# Autodesk Inventor assembly: Arm Assembly
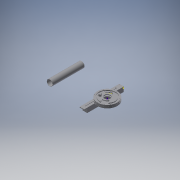
[picture p0: Inventor's stored thumbnail of the model, 180x180]
Saved by Autodesk Inventor 2016 (Build 200138000, 138)
## iProperties
Created: 2016-04-23
Part Number: Arm Assembly
Document SubType Name: Assembly
Designer: rubenjm
Author: rubenjm
## Documents named in this file (22)
- C:\Users\rubenjm\Documents\To Transfer\2k16 Spring\RME\GGC\V3\Arm Assembly.iam
- C:\Users\rubenjm\Documents\To Transfer\2k16 Spring\RME\GGC\V3\Inner Pole.ipt
- C:\Users\rubenjm\Documents\To Transfer\2k16 Spring\RME\GGC\V3\Arm Base.ipt
- C:\Users\rubenjm\Documents\To Transfer\2k16 Spring\RME\GGC\V3\Holder.ipt
- C:\Users\rubenjm\Documents\To Transfer\2k16 Spring\RME\GGC\V3\Threaded Rod Nut.ipt
- C:\Users\rubenjm\Documents\To Transfer\2k16 Spring\RME\GGC\V3\Unthreaded Rod.ipt
- C:\Users\rubenjm\Documents\To Transfer\2k16 Spring\RME\GGC\V3\Threaded Rod.ipt
- C:\Users\rubenjm\Documents\To Transfer\2k16 Spring\RME\GGC\V3\NEMA23 Motor.ipt
- C:\Users\rubenjm\Documents\To Transfer\2k16 Spring\RME\GGC\V3\Motor Coupler.ipt
- C:\Users\rubenjm\Documents\To Transfer\2k16 Spring\RME\GGC\V3\Far End Cap.ipt
- C:\Users\rubenjm\Documents\To Transfer\2k16 Spring\RME\GGC\V3\Near Holder.ipt
- C:\Users\rubenjm\Documents\To Transfer\2k16 Spring\RME\GGC\V3\Motor Bracket.ipt
- C:\Users\rubenjm\Documents\To Transfer\2k16 Spring\RME\GGC\V3\Near End Cap.ipt
- C:\Users\rubenjm\Documents\To Transfer\2k16 Spring\RME\GGC\V3\Arm Side.ipt
- C:\Users\rubenjm\Documents\To Transfer\2k16 Spring\RME\GGC\V3\Arm Top.ipt
- C:\Users\rubenjm\Documents\To Transfer\2k16 Spring\RME\GGC\V3\Turntable Top.ipt
- C:\Users\rubenjm\Documents\To Transfer\2k16 Spring\RME\GGC\V3\Turntable.ipt
- C:\Users\rubenjm\Documents\To Transfer\2k16 Spring\RME\GGC\V3\Turntable Ring Gear.iam
- C:\Users\rubenjm\Documents\To Transfer\2k16 Spring\RME\GGC\V3\Turntable Sheath.ipt
- C:\Users\rubenjm\Documents\To Transfer\2k16 Spring\RME\GGC\V3\NEMA16 Motor.ipt
- C:\Users\rubenjm\Documents\To Transfer\2k16 Spring\RME\GGC\V3\Turntable Mount.ipt
- C:\Users\rubenjm\Documents\To Transfer\2k16 Spring\RME\GGC\V3\Inner Gear.iam
## Components (28 placed, 21 different names)
1. Inner Pole:1
2. Arm Base:1 — Mate:1, Mate:2, Mate:15, Mate:26, Mate:27, Flush:1, Flush:3, Mate:34, Mate:38, Flush:4, Mate:40, Flush:5, Mate:41, Mate:42, Mate:43, Flush:6, Flush:7, Flush:9, Flush:11, Mate:48
3. Holder:1 — Mate:1, Mate:2, Mate:8, Mate:9, Mate:10, Mate:12, Mate:13, Mate:49
4. Holder:2 — Mate:15, Mate:16, Mate:17, Mate:18, Mate:19, Mate:20, Mate:46, Mate:47, Mate:51
5. Threaded Rod Nut:1 — Mate:8, Mate:9, Mate:10, Mate:11
6. Threaded Rod Nut:2 — Mate:18, Mate:19, Mate:20
7. Unthreaded Rod:1 — Mate:13, Mate:16, Mate:28
8. Unthreaded Rod:2 — Mate:12, Mate:17, Mate:29
9. Threaded Rod:1 — Mate:11, Mate:24, Mate:25, Mate:30
10. NEMA23 Motor:1 — Mate:35, Mate:36, Mate:37, Mate:39
11. Motor Coupler:1 — Mate:24, Mate:25
12. Far End Cap:1 — Mate:26, Mate:27, Flush:1, Mate:28, Mate:29, Mate:30, Mate:44, Flush:12
13. Near Holder:1 — Flush:5, Mate:41, Mate:42
14. Motor Bracket:1 — Flush:3, Mate:34, Mate:35, Mate:36, Mate:37, Mate:38
15. Near End Cap:1 — Mate:39, Flush:4, Mate:40, Flush:8, Flush:10
16. Arm Side:1 — Mate:43, Flush:6, Flush:7, Flush:8
17. Arm Side:2 — Flush:9, Flush:10, Flush:11, Mate:45
18. Arm Top:1 — Mate:44, Mate:45, Flush:12
19. Turntable Top:1 — Mate:46, Mate:47, Mate:48, Mate:49, Mate:50, Mate:53
20. Turntable:1 — Mate:60, Mate:61, Mate:62, Mate:69, Mate:70, Mate:71
21. Turntable Top:2 — Mate:50, Mate:51, Mate:53, Mate:54, Mate:55, Mate:56
22. Turntable Ring Gear:1 [sub-assembly] — Mate:54, Mate:55, Mate:56, Mate:57, Mate:58, Mate:59, Mate:62
23. Turntable Ring Gear:2 [sub-assembly] — Mate:57, Mate:58, Mate:59, Mate:60, Mate:61, Mate:63, Mate:64, Mate:65
24. Turntable Sheath:1 — Mate:66, Mate:67, Mate:68
25. Turntable Sheath:2 — Mate:63, Mate:64, Mate:65, Mate:66, Mate:67, Mate:68
26. NEMA16 Motor:1 — Mate:72, Mate:73, Mate:74, Mate:75, Mate:76
27. Turntable Mount:1 — Mate:69, Mate:70, Mate:71, Mate:72, Mate:73, Mate:74
28. Inner Gear:1 [sub-assembly] — Mate:75, Mate:76
## Relationships (74: Mate 63, Flush 11)
- Mate:1: Arm Base:1 ↔ Holder:1
- Mate:2: Arm Base:1 ↔ Holder:1
- Mate:8: Holder:1 ↔ Threaded Rod Nut:1
- Mate:9: Holder:1 ↔ Threaded Rod Nut:1
- Mate:10: Holder:1 ↔ Threaded Rod Nut:1
- Mate:11: Threaded Rod Nut:1 ↔ Threaded Rod:1
- Mate:12: Holder:1 ↔ Unthreaded Rod:2
- Mate:13: Holder:1 ↔ Unthreaded Rod:1
- Mate:15: Arm Base:1 ↔ Holder:2
- Mate:16: Holder:2 ↔ Unthreaded Rod:1
- Mate:17: Holder:2 ↔ Unthreaded Rod:2
- Mate:18: Holder:2 ↔ Threaded Rod Nut:2
- Mate:19: Holder:2 ↔ Threaded Rod Nut:2
- Mate:20: Holder:2 ↔ Threaded Rod Nut:2
- Mate:24: Threaded Rod:1 ↔ Motor Coupler:1
- Mate:25: Threaded Rod:1 ↔ Motor Coupler:1
- Mate:26: Arm Base:1 ↔ Far End Cap:1
- Mate:27: Arm Base:1 ↔ Far End Cap:1
- Flush:1: Arm Base:1 ↔ Far End Cap:1
- Mate:28: Unthreaded Rod:1 ↔ Far End Cap:1
- Mate:29: Unthreaded Rod:2 ↔ Far End Cap:1
- Mate:30: Threaded Rod:1 ↔ Far End Cap:1
- Flush:3: Arm Base:1 ↔ Motor Bracket:1
- Mate:34: Arm Base:1 ↔ Motor Bracket:1
- Mate:35: NEMA23 Motor:1 ↔ Motor Bracket:1
- Mate:36: NEMA23 Motor:1 ↔ Motor Bracket:1
- Mate:37: NEMA23 Motor:1 ↔ Motor Bracket:1
- Mate:38: Arm Base:1 ↔ Motor Bracket:1
- Mate:39: NEMA23 Motor:1 ↔ Near End Cap:1
- Flush:4: Arm Base:1 ↔ Near End Cap:1
- Mate:40: Arm Base:1 ↔ Near End Cap:1
- Flush:5: Arm Base:1 ↔ Near Holder:1
- Mate:41: Arm Base:1 ↔ Near Holder:1
- Mate:42: Arm Base:1 ↔ Near Holder:1
- Mate:43: Arm Base:1 ↔ Arm Side:1
- Flush:6: Arm Base:1 ↔ Arm Side:1
- Flush:7: Arm Base:1 ↔ Arm Side:1
- Flush:8: Near End Cap:1 ↔ Arm Side:1
- Flush:9: Arm Base:1 ↔ Arm Side:2
- Flush:10: Near End Cap:1 ↔ Arm Side:2
- Flush:11: Arm Base:1 ↔ Arm Side:2
- Mate:44: Far End Cap:1 ↔ Arm Top:1
- Mate:45: Arm Side:2 ↔ Arm Top:1
- Flush:12: Far End Cap:1 ↔ Arm Top:1
- Mate:46: Holder:2 ↔ Turntable Top:1
- Mate:47: Holder:2 ↔ Turntable Top:1
- Mate:48: Arm Base:1 ↔ Turntable Top:1
- Mate:49: Holder:1 ↔ Turntable Top:1
- Mate:50: Turntable Top:1 ↔ Turntable Top:2
- Mate:51: Holder:2 ↔ Turntable Top:2
- Mate:53: Turntable Top:1 ↔ Turntable Top:2
- Mate:54: Turntable Top:2 ↔ Turntable Ring Gear:1
- Mate:55: Turntable Top:2 ↔ Turntable Ring Gear:1
- Mate:56: Turntable Top:2 ↔ Turntable Ring Gear:1
- Mate:57: Turntable Ring Gear:1 ↔ Turntable Ring Gear:2
- Mate:58: Turntable Ring Gear:1 ↔ Turntable Ring Gear:2
- Mate:59: Turntable Ring Gear:1 ↔ Turntable Ring Gear:2
- Mate:60: Turntable:1 ↔ Turntable Ring Gear:2
- Mate:61: Turntable:1 ↔ Turntable Ring Gear:2
- Mate:62: Turntable:1 ↔ Turntable Ring Gear:1
- Mate:63: Turntable Ring Gear:2 ↔ Turntable Sheath:2
- Mate:64: Turntable Ring Gear:2 ↔ Turntable Sheath:2
- Mate:65: Turntable Ring Gear:2 ↔ Turntable Sheath:2
- Mate:66: Turntable Sheath:1 ↔ Turntable Sheath:2
- Mate:67: Turntable Sheath:1 ↔ Turntable Sheath:2
- Mate:68: Turntable Sheath:1 ↔ Turntable Sheath:2
- Mate:69: Turntable:1 ↔ Turntable Mount:1
- Mate:70: Turntable:1 ↔ Turntable Mount:1
- Mate:71: Turntable:1 ↔ Turntable Mount:1
- Mate:72: NEMA16 Motor:1 ↔ Turntable Mount:1
- Mate:73: NEMA16 Motor:1 ↔ Turntable Mount:1
- Mate:74: NEMA16 Motor:1 ↔ Turntable Mount:1
- Mate:75: NEMA16 Motor:1 ↔ Inner Gear:1
- Mate:76: NEMA16 Motor:1 ↔ Inner Gear:1
